# Autodesk Inventor assembly: ウイング1
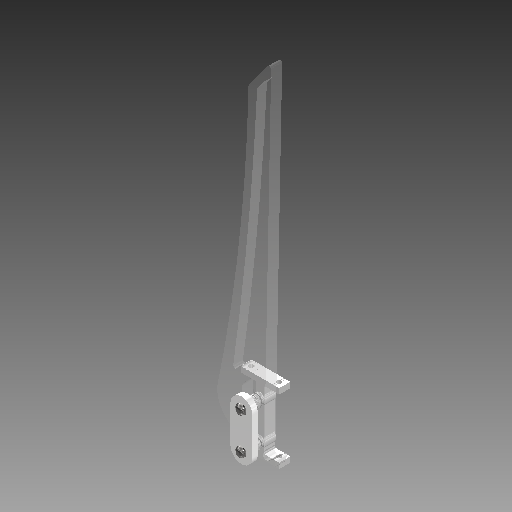
[picture p0: Inventor's stored thumbnail of the model, 512x512]
Saved by Autodesk Inventor 2020 (Build 240168000, 168)
## iProperties
Created: 2019-09-04
Part Number: ウイング1
Document SubType Name: Assembly
Designer: 雪村
Mass: 23.2611 g
Surface Area: 136.785 cm^2
Volume: 15.202 cm^3
Density: 1.53013 g/cm^3
Author: 雪村
## Documents named in this file (6)
- C:\Users\white\Documents\SRDC\SRDC\Inventor_2017\2018年機体\2020年4年機体\ウイング1.iam
- C:\Users\white\Documents\SRDC\SRDC\Inventor_2017\2018年機体\2020年4年機体\ウイング土台2.ipt
- C:\Users\white\Documents\SRDC\SRDC\Inventor_2017\2018年機体\パーツ\スペーサーm3,7.ipt
- C:\Users\white\Documents\SRDC\SRDC\Inventor_2017\2018年機体\2020年4年機体\ウイング1.ipt
- C:\Users\white\Documents\SRDC\SRDC\Inventor_2017\2018年機体\alternative\ウイング抑え1.ipt
- C:\Users\white\Documents\SRDC\SRDC\Inventor_2017\2018年機体\パーツ\ネジ鍋m3,16.ipt
## Components (7 placed, 5 different names)
1. ウイング土台2:1 — 挿入:1, 挿入:2
2. スペーサーm3,7:1 — 挿入:1, 挿入:3
3. スペーサーm3,7:2 — 挿入:2, フラッシュ:1, 挿入:4, メイト:1
4. ウイング1:1 — フラッシュ:1, メイト:1
5. ウイング抑え1:1 — 挿入:3, 挿入:4, 挿入:5, 挿入:6
6. ネジ鍋m3,16:1 — 挿入:5
7. ネジ鍋m3,16:2 — 挿入:6
## Relationships (8: Insert 6, Flush 1, Mate 1)
- 挿入:1 [Insert]: ウイング土台2:1 ↔ スペーサーm3,7:1
- 挿入:2 [Insert]: ウイング土台2:1 ↔ スペーサーm3,7:2
- フラッシュ:1 [Flush] (-0.5 mm): スペーサーm3,7:2 ↔ ウイング1:1
- 挿入:3 [Insert]: スペーサーm3,7:1 ↔ ウイング抑え1:1
- 挿入:4 [Insert]: スペーサーm3,7:2 ↔ ウイング抑え1:1
- 挿入:5 [Insert]: ウイング抑え1:1 ↔ ネジ鍋m3,16:1
- 挿入:6 [Insert]: ウイング抑え1:1 ↔ ネジ鍋m3,16:2
- メイト:1 [Mate]: スペーサーm3,7:2 ↔ ウイング1:1
